# Autodesk Inventor assembly: shield2
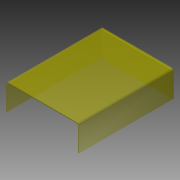
[picture p0: Inventor's stored thumbnail of the model, 180x180]
Saved by Autodesk Inventor 2014 SP2 (Build 180246200, 246)
## iProperties
Created: 2016-10-05
Part Number: shield2
Document SubType Name: Assembly
Designer: cruiser
Author: cruiser
## Documents named in this file (3)
- C:\Users\cruiser\Desktop\models\3d printers\laserresin5\shield2.iam
- C:\Users\cruiser\Desktop\models\3d printers\laserresin5\shield2a.ipt
- C:\Users\cruiser\Desktop\models\3d printers\laserresin5\shield2b.ipt
## Components (2 placed, 2 different names)
1. shield2a:1 — Mate:1, Mate:2, Flush:1
2. shield2b:1 — Mate:1, Mate:2, Flush:1
## Relationships (3: Mate 2, Flush 1)
- Mate:1: shield2a:1 ↔ shield2b:1
- Mate:2: shield2a:1 ↔ shield2b:1
- Flush:1: shield2a:1 ↔ shield2b:1
